# Autodesk Inventor assembly: rapoukBaseAssemblyv1
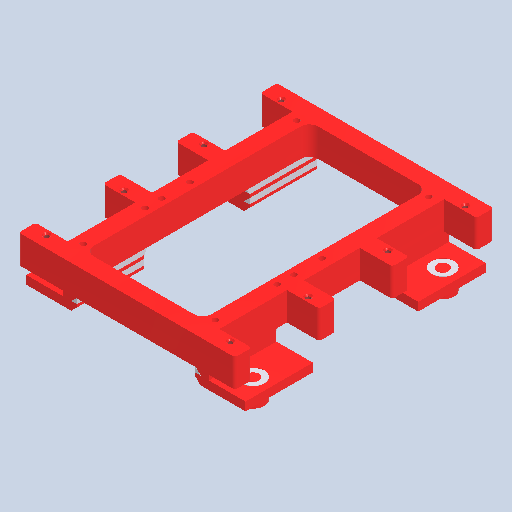
[picture p0: Inventor's stored thumbnail of the model, 512x512]
Saved by Autodesk Inventor 2024 (Build 280153000, 153)
## iProperties
Created: 2024-02-06
Part Number: rapoukBaseAssemblyv1
Document SubType Name: Weldment
Designer: Roman Suk
Weld Material: Welded Aluminum-6061
Author: Roman Suk
## Documents named in this file (5)
- C:\Users\Roman Suk\Documents\Ročníkovka SŠ\Technical documentation\Final1\rapoukBaseAssemblyv1.iam
- C:\Users\Roman Suk\Documents\Ročníkovka SŠ\Technical documentation\Final1\rapoukBasev5.ipt
- C:\Users\Roman Suk\Documents\Ročníkovka SŠ\Technical documentation\Final1\rapoukLegBasev3.ipt
- C:\Users\Roman Suk\Documents\Ročníkovka SŠ\Technical documentation\Final1\rapoukLegSupportv1.ipt
- C:\Users\Roman Suk\Documents\Ročníkovka SŠ\Technical documentation\Final1\rapoukLegPinv1.ipt
## Components (13 placed, 4 different names)
1. rapoukBasev5:1 — Mate:1, Mate:2, Mate:3, Mate:4, Flush:1, Flush:2, Flush:3, Flush:4, Flush:5, Flush:6, Flush:7, Flush:8
2. rapoukLegBasev3:1 — Insert:4, Mate:7, Flush:13, Flush:14
3. rapoukLegBasev3:2 — Mate:6, Flush:16, Insert:5, Flush:17
4. rapoukLegBasev3:4 — Insert:3, Flush:12, Flush:15, Mate:8
5. rapoukLegSupportv1:1 — Mate:1, Flush:4, Flush:8, Mate:7, Flush:13, Flush:14
6. rapoukLegSupportv1:2 — Mate:2, Flush:1, Flush:7, Flush:18, Flush:19, Mate:9
7. rapoukLegSupportv1:3 — Mate:3, Flush:2, Flush:6, Mate:6, Flush:16, Flush:17
8. rapoukLegSupportv1:4 — Mate:4, Flush:3, Flush:5, Flush:12, Flush:15, Mate:8
9. rapoukLegPinv1:1 — Insert:5
10. rapoukLegPinv1:3 — Insert:3
11. rapoukLegPinv1:4 — Insert:4
12. rapoukLegPinv1:5 — Insert:6
13. rapoukLegBasev3:5 — Insert:6, Flush:18, Flush:19, Mate:9
## Relationships (28: Flush 16, Mate 8, Insert 4)
- Insert:3: rapoukLegBasev3:4 ↔ rapoukLegPinv1:3
- Insert:4: rapoukLegBasev3:1 ↔ rapoukLegPinv1:4
- Mate:1: rapoukBasev5:1 ↔ rapoukLegSupportv1:1
- Mate:2: rapoukBasev5:1 ↔ rapoukLegSupportv1:2
- Mate:3: rapoukBasev5:1 ↔ rapoukLegSupportv1:3
- Mate:4: rapoukBasev5:1 ↔ rapoukLegSupportv1:4
- Flush:1: rapoukBasev5:1 ↔ rapoukLegSupportv1:2
- Flush:2: rapoukBasev5:1 ↔ rapoukLegSupportv1:3
- Flush:3: rapoukBasev5:1 ↔ rapoukLegSupportv1:4
- Flush:4: rapoukBasev5:1 ↔ rapoukLegSupportv1:1
- Flush:5 (-3.25 mm): rapoukBasev5:1 ↔ rapoukLegSupportv1:4
- Flush:6 (-3.25 mm): rapoukBasev5:1 ↔ rapoukLegSupportv1:3
- Flush:7 (3.25 mm): rapoukBasev5:1 ↔ rapoukLegSupportv1:2
- Flush:8 (3.25 mm): rapoukBasev5:1 ↔ rapoukLegSupportv1:1
- Mate:6: rapoukLegBasev3:2 ↔ rapoukLegSupportv1:3
- Mate:7: rapoukLegBasev3:1 ↔ rapoukLegSupportv1:1
- Flush:12: rapoukLegBasev3:4 ↔ rapoukLegSupportv1:4
- Flush:13: rapoukLegBasev3:1 ↔ rapoukLegSupportv1:1
- Flush:14: rapoukLegBasev3:1 ↔ rapoukLegSupportv1:1
- Flush:15: rapoukLegBasev3:4 ↔ rapoukLegSupportv1:4
- Flush:16: rapoukLegBasev3:2 ↔ rapoukLegSupportv1:3
- Mate:8: rapoukLegBasev3:4 ↔ rapoukLegSupportv1:4
- Insert:5: rapoukLegBasev3:2 ↔ rapoukLegPinv1:1
- Flush:17: rapoukLegBasev3:2 ↔ rapoukLegSupportv1:3
- Insert:6: rapoukLegPinv1:5 ↔ rapoukLegBasev3:5
- Flush:18: rapoukLegSupportv1:2 ↔ rapoukLegBasev3:5
- Flush:19: rapoukLegSupportv1:2 ↔ rapoukLegBasev3:5
- Mate:9: rapoukLegSupportv1:2 ↔ rapoukLegBasev3:5
